# Autodesk Inventor assembly: sg90 long claw
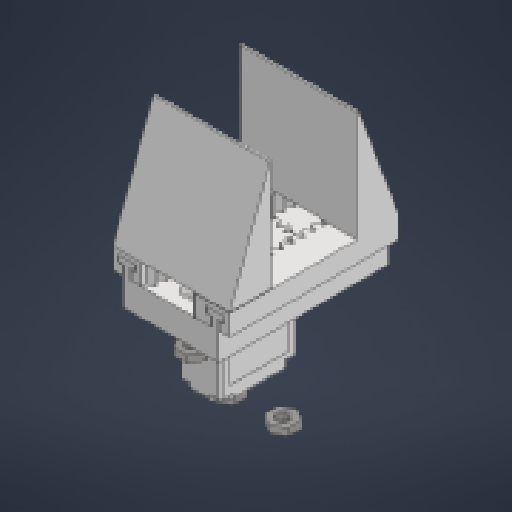
[picture p0: Inventor's stored thumbnail of the model, 512x512]
Saved by Autodesk Inventor 2026.2 (Build 302298000, 298)
## iProperties
Created: 2025-06-09
Part Number: sg90 long claw
Document SubType Name: Assembly
Designer: gavin
Author: gavin
## Documents named in this file (9)
- D:\Github\6-DOF-Robot-Arm\3D-model\robot armT 2(CAD file)\sg90 long claw.iam
- D:\Github\6-DOF-Robot-Arm\3D-model\robot armT 2(CAD file)\9G Servo Motor SG90.ipt
- D:\Github\6-DOF-Robot-Arm\3D-model\robot armT 2(CAD file)\sg90 claw v2.ipt
- D:\Github\6-DOF-Robot-Arm\3D-model\robot armT 2(CAD file)\sg90 claw v2 gear m1.ipt
- D:\Github\6-DOF-Robot-Arm\3D-model\robot armT 2(CAD file)\sg90 claw v2 holder.ipt
- D:\Github\6-DOF-Robot-Arm\3D-model\robot armT 2(CAD file)\sg90 claw finger long.ipt
- C:\Users\gavin\Documents\Inventor\Content Center Files\R2026\en-US\ASME ANSI B18.3.5M(2)\ASME_ANSI B18.3.5M - M3x10(2).ipt
- D:\Github\6-DOF-Robot-Arm\3D-model\robot armT 2(CAD file)\AS 1474 - M4(1).ipt
- C:\Users\gavin\Documents\Inventor\Content Center Files\R2026\en-US\IS 7483\IS 7483 - M3 x 14.ipt
## Components (14 placed, 8 different names)
1. 9G Servo Motor SG90:1 — 貼合:8, 貼合:9, 貼合:10
2. sg90 claw v2:1 — 貼合:10, 齊平:3, 齊平:4, 剛性:7, 剛性:8
3. sg90 claw v2 gear m1:1
4. sg90 claw v2 holder:1 — 貼合:8, 貼合:9, 剛性:1, 剛性:2, 剛性:5, 剛性:6
5. sg90 claw finger long:1 — 齊平:3
6. sg90 claw finger long:2 — 齊平:4
7. Broached Hexagon Socket Flat Countersunk Head Cap Screws - Metric M3x10:1 — 剛性:2, 剛性:4
8. Broached Hexagon Socket Flat Countersunk Head Cap Screws - Metric M3x10:2 — 剛性:1, 剛性:3
9. AS 1474 - M4(1):1 — 剛性:3
10. AS 1474 - M4(1):2 — 剛性:4
11. AS 1474 - M4(1):3 — 剛性:6
12. IS 7483 M3 x 14:1 — 剛性:7
13. AS 1474 - M4(1):4 — 剛性:5
14. IS 7483 M3 x 14:2 — 剛性:8
## Relationships (22: Mate 10, WeldJoint 8, Flush 4)
- [Flush]: 9G Servo Motor SG90:1 ↔ sg90 claw v2:1
- [Mate]: 9G Servo Motor SG90:1 ↔ sg90 claw v2 gear m1:1
- [Mate]: 9G Servo Motor SG90:1 ↔ sg90 claw v2 gear m1:1
- [Mate]: 9G Servo Motor SG90:1 ↔ sg90 claw v2:1
- [Flush]: 9G Servo Motor SG90:1 ↔ sg90 claw v2 holder:1
- [Mate]: sg90 claw v2:1 ↔ sg90 claw finger long:1
- [Mate] (0.2 mm): sg90 claw v2:1 ↔ sg90 claw finger long:1
- [Mate]: sg90 claw v2:1 ↔ sg90 claw finger long:2
- [Mate] (0.2 mm): sg90 claw v2:1 ↔ sg90 claw finger long:2
- 貼合:8 [Mate]: 9G Servo Motor SG90:1 ↔ sg90 claw v2 holder:1
- 貼合:9 [Mate]: 9G Servo Motor SG90:1 ↔ sg90 claw v2 holder:1
- 貼合:10 [Mate]: 9G Servo Motor SG90:1 ↔ sg90 claw v2:1
- 齊平:3 [Flush]: sg90 claw v2:1 ↔ sg90 claw finger long:1
- 齊平:4 [Flush]: sg90 claw v2:1 ↔ sg90 claw finger long:2
- 剛性:1 [WeldJoint]: sg90 claw v2 holder:1 ↔ Broached Hexagon Socket Flat Countersunk Head Cap Screws - Metric M3x10:2
- 剛性:2 [WeldJoint]: sg90 claw v2 holder:1 ↔ Broached Hexagon Socket Flat Countersunk Head Cap Screws - Metric M3x10:1
- 剛性:3 [WeldJoint]: Broached Hexagon Socket Flat Countersunk Head Cap Screws - Metric M3x10:2 ↔ AS 1474 - M4(1):1
- 剛性:4 [WeldJoint]: Broached Hexagon Socket Flat Countersunk Head Cap Screws - Metric M3x10:1 ↔ AS 1474 - M4(1):2
- 剛性:5 [WeldJoint]: sg90 claw v2 holder:1 ↔ AS 1474 - M4(1):4
- 剛性:6 [WeldJoint]: sg90 claw v2 holder:1 ↔ AS 1474 - M4(1):3
- 剛性:7 [WeldJoint]: sg90 claw v2:1 ↔ IS 7483 M3 x 14:1
- 剛性:8 [WeldJoint]: sg90 claw v2:1 ↔ IS 7483 M3 x 14:2
